# Autodesk Inventor assembly: Shooter Assembly v2
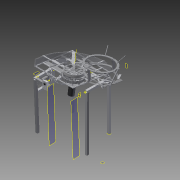
[picture p0: Inventor's stored thumbnail of the model, 180x180]
Saved by Autodesk Inventor 2013 (Build 170138000, 138)
## iProperties
Created: 2013-01-15
Part Number: Shooter Assembly v2
Document SubType Name: Assembly
Designer: actoennies
Mass: 8056.1 g
Surface Area: 23883.9 cm^2
Volume: 3889.96 cm^3
Density: 2.071 g/cm^3
Author: actoennies
## Documents named in this file (34)
- \\NNHSSRV2.hs.sd203.org\ACToennies$\Robotics\Shooter\Shooter Assembly v2.iam
- \\NNHSSRV2.hs.sd203.org\ACToennies$\Robotics\Shooter\Bearing Mount v1.ipt
- \\NNHSSRV2.hs.sd203.org\ACToennies$\Robotics\Shooter\Outer Rail v1.ipt
- \\NNHSSRV2.hs.sd203.org\ACToennies$\Robotics\Shooter\Runner Rails v2.ipt
- \\NNHSSRV2.hs.sd203.org\ACToennies$\Robotics\Shooter\Bearing.ipt
- \\NNHSSRV2.hs.sd203.org\ACToennies$\Robotics\Shooter\Flywheel Assembly.iam
- \\NNHSSRV2.hs.sd203.org\ACToennies$\Robotics\Shooter\Shooter Mounter.ipt
- \\NNHSSRV2.hs.sd203.org\ACToennies$\Robotics\Shooter\Bearing Mount 2 v1.ipt
- \\NNHSSRV2.hs.sd203.org\ACToennies$\Robotics\Shooter\Shorter Shaft.ipt
- \\NNHSSRV2.hs.sd203.org\ACToennies$\Robotics\Shooter\Spacer Rube.ipt
- \\NNHSSRV2.hs.sd203.org\ACToennies$\Robotics\Shooter\Edge Mount.ipt
- \\NNHSSRV2.hs.sd203.org\ACToennies$\Robotics\Shooter\Tower Corner Mount.ipt
- \\NNHSSRV2.hs.sd203.org\ACToennies$\Robotics\Shooter\Square Tube.ipt
- \\NNHSSRV2.hs.sd203.org\ACToennies$\Robotics\Shooter\Flange Bearing Mount Tower.ipt
- \\NNHSSRV2.hs.sd203.org\ACToennies$\Robotics\Shooter\Flange Bearing Mount Tower Mirror.ipt
- \\NNHSSRV2.hs.sd203.org\ACToennies$\Robotics\Shooter\Bearing Mount Top.ipt
- \\NNHSSRV2.hs.sd203.org\ACToennies$\Robotics\Shooter\Square Motor Mount.ipt
- \\NNHSSRV2.hs.sd203.org\ACToennies$\Robotics\Hopper\HopperAssembly42inch_v5.iam
- \\NNHSSRV2.hs.sd203.org\ACToennies$\Robotics\Shooter\Shooter Assembly v2\Design Accelerator\Spur Gears1.iam
- \\NNHSSRV2.hs.sd203.org\ACToennies$\Robotics\Parts\Imported Components\Snow Blower Motor\Snow Blower Motor.iam
- \\NNHSSRV2.hs.sd203.org\ACToennies$\Robotics\Shooter\Snowblower Motor Mount.ipt
- \\NNHSSRV2.hs.sd203.org\ACToennies$\Robotics\Shooter\Edge Mount Interference.ipt
- \\NNHSSRV2.hs.sd203.org\ACToennies$\Robotics\Shooter\8mm shaft.ipt
- \\NNHSSRV2.hs.sd203.org\ACToennies$\Robotics\Shooter\CIM Bearing.ipt
- H:\Robotics\Parts\8 Plaction Wheel.iam
- \\NNHSSRV2.hs.sd203.org\ACToennies$\Robotics\Shooter\Square Tube 2.ipt
- \\NNHSSRV2.hs.sd203.org\ACToennies$\Robotics\Parts\CIM Motor\Motors_FR801-001.iam
- \\NNHSSRV2.hs.sd203.org\ACToennies$\Robotics\Shooter\Cim Mount.ipt
- \\NNHSSRV2.hs.sd203.org\ACToennies$\Robotics\Shooter\Hub v1.ipt
- \\NNHSSRV2.hs.sd203.org\ACToennies$\Robotics\Shooter\Camera Traffic Light Mount.ipt
- \\NNHSSRV2.hs.sd203.org\ACToennies$\Robotics\Shooter\Camera Gusset Plat.ipt
- \\NNHSSRV2.hs.sd203.org\ACToennies$\Inventor\Camera.ipt
- \\NNHSSRV2.hs.sd203.org\ACToennies$\Robotics\Shooter\Square Tube 3.ipt
- \\NNHSSRV2.hs.sd203.org\ACToennies$\Robotics\Shooter\Square Tube 4.ipt
## Components (40 placed, 33 different names)
1. Bearing Mount v1:1 — Insert:12, Insert:13, Insert:14, Insert:15, Insert:26, Insert:27, Mate:62, Mate:63
2. Outer Rail v1:1 — Insert:12, Insert:13, Insert:47, Insert:48, Flush:21, Mate:87
3. Runner Rails v2:1 — Insert:14, Insert:15, Mate:42
4. Flywheel Assembly:1 [sub-assembly] — Mate:61, Flush:30, Mate:68, Flush:31
5. Shooter Mounter:1 — Insert:26, Insert:27, Insert:34, Flush:11, Insert:35, Insert:36, Insert:37, Insert:38, Flush:19, Mate:45, Flush:24, Flush:40
6. Spacer Rube:1 — Insert:34, Flush:11
7. Bearing Mount 2 v1:1 — Insert:37, Insert:38, Insert:40
8. Bearing Mount 2 v1:2 — Insert:35, Insert:36, Insert:39
9. Bearing:3 — Insert:40, Flush:13, Mate:14, Mate:15
10. Bearing:4 — Insert:39, Flush:12, Mate:12, Mate:13, Mate:36, Mate:44
11. Shorter Shaft:1 — Flush:12, Mate:12, Mate:13, Mate:37
12. Shorter Shaft:2 — Flush:13, Mate:14, Mate:15, Mate:38
13. Tower Corner Mount:1 — Mate:16, Flush:14, Mate:48, Flush:33
14. Edge Mount:2 — Flush:34, Mate:104, Flush:48, Mate:105, Mate:106, Flush:50
15. Square Tube:2 — Mate:16, Flush:14, Insert:41, Insert:42, Flush:19, Flush:23, Flush:26, Mate:50, Mate:52, Flush:27, Mate:81, Flush:32, Mate:93, Flush:41, Flush:42
16. Flange Bearing Mount Tower:1 — Insert:41, Insert:42, Insert:43
17. Bearing:5 — Insert:43, Mate:36, Mate:37
18. Flange Bearing Mount Tower Mirror:1 — Insert:46, Flush:29
19. Bearing:6 — Insert:46, Mate:38
20. Bearing Mount Top:1 — Insert:47, Insert:48, Mate:65, Mate:66, Mate:68
21. Square Motor Mount:1 — Flush:23, Mate:47, Mate:48, Mate:51, Flush:27, Mate:77
22. HopperAssembly42inch_v5:1 [sub-assembly] — Mate:42, Flush:21, Mate:87
23. Spur Gears:1 [sub-assembly] — Mate:44, Mate:45, Flush:24, Flush:25, Mate:46, Angle:2
24. Snow Blower Motor:1 [sub-assembly] — Flush:25, Mate:46, Angle:2, Insert:50, Insert:51
25. Snowblower Motor Mount:1 — Insert:50, Insert:51, Mate:47, Mate:51, Mate:52
26. Edge Mount Interference:1 — Flush:26, Mate:50, Mate:77, Mate:95, Flush:44, Flush:45, Flush:46
27. 8mm shaft:1 — Mate:61, Flush:30, Mate:67, Flush:31, Mate:82, Mate:83, Mate:84, Mate:86
28. CIM Bearing:1 — Mate:65, Mate:66, Mate:67
29. CIM Bearing:2 — Mate:62, Mate:63, Insert:56
30. 8 Plaction Wheel:1 [sub-assembly] — Mate:88, Mate:89, Mate:90, Mate:91, Mate:92
31. Square Tube 2:1 — Mate:81, Flush:32, Flush:33, Flush:34, Mate:106, Mate:107
32. Motors_FR801-001:1 [sub-assembly] — Mate:82, Mate:83, Mate:84, Insert:58
33. Cim Mount:1 — Insert:58, Flush:40
34. Hub v1:1 — Mate:88, Mate:89, Mate:90, Flush:38
35. Hub v1:2 — Mate:91, Flush:38, Mate:92, Insert:56
36. Camera Traffic Light Mount:1 — Mate:93, Flush:41, Flush:42, Mate:94, Flush:43, Mate:101, Mate:102, Mate:103
37. Camera Gusset Plat:1 — Mate:94, Mate:95, Flush:43
38. Camera:1 — Mate:101, Mate:102, Mate:103
39. Square Tube 3:1 — Mate:104, Flush:48, Mate:105, Mate:107, Mate:109, Mate:110, Mate:112, Mate:113, Mate:117, Mate:121
40. Square Tube 4:1 — Mate:114, Mate:115, Mate:116, Mate:117, Mate:119, Mate:121
## Relationships (108: Mate 57, Flush 27, Insert 23, Angle 1)
- Insert:12: Bearing Mount v1:1 ↔ Outer Rail v1:1
- Insert:13: Bearing Mount v1:1 ↔ Outer Rail v1:1
- Insert:14: Bearing Mount v1:1 ↔ Runner Rails v2:1
- Insert:15: Bearing Mount v1:1 ↔ Runner Rails v2:1
- Insert:26: Bearing Mount v1:1 ↔ Shooter Mounter:1
- Insert:27: Bearing Mount v1:1 ↔ Shooter Mounter:1
- Insert:34: Shooter Mounter:1 ↔ Spacer Rube:1
- Flush:11: Shooter Mounter:1 ↔ Spacer Rube:1
- Insert:35: Shooter Mounter:1 ↔ Bearing Mount 2 v1:2
- Insert:36: Shooter Mounter:1 ↔ Bearing Mount 2 v1:2
- Insert:37: Shooter Mounter:1 ↔ Bearing Mount 2 v1:1
- Insert:38: Shooter Mounter:1 ↔ Bearing Mount 2 v1:1
- Insert:39: Bearing Mount 2 v1:2 ↔ Bearing:4
- Insert:40: Bearing Mount 2 v1:1 ↔ Bearing:3
- Flush:12 (-25.4 mm): Bearing:4 ↔ Shorter Shaft:1
- Mate:12: Bearing:4 ↔ Shorter Shaft:1
- Mate:13: Bearing:4 ↔ Shorter Shaft:1
- Flush:13 (-25.4 mm): Bearing:3 ↔ Shorter Shaft:2
- Mate:14: Bearing:3 ↔ Shorter Shaft:2
- Mate:15: Bearing:3 ↔ Shorter Shaft:2
- Mate:16: Tower Corner Mount:1 ↔ Square Tube:2
- Flush:14: Tower Corner Mount:1 ↔ Square Tube:2
- Insert:41: Square Tube:2 ↔ Flange Bearing Mount Tower:1
- Insert:42: Square Tube:2 ↔ Flange Bearing Mount Tower:1
- Insert:43: Flange Bearing Mount Tower:1 ↔ Bearing:5
- Flush:19: Shooter Mounter:1 ↔ Square Tube:2
- Mate:36: Bearing:4 ↔ Bearing:5
- Mate:37: Shorter Shaft:1 ↔ Bearing:5
- Insert:46: Flange Bearing Mount Tower Mirror:1 ↔ Bearing:6
- Mate:38: Shorter Shaft:2 ↔ Bearing:6
- Insert:47: Outer Rail v1:1 ↔ Bearing Mount Top:1
- Insert:48: Outer Rail v1:1 ↔ Bearing Mount Top:1
- Mate:42: Runner Rails v2:1 ↔ HopperAssembly42inch_v5:1
- Flush:21: Outer Rail v1:1 ↔ HopperAssembly42inch_v5:1
- Flush:23 (152.4 mm): Square Tube:2 ↔ Square Motor Mount:1
- Mate:44: Bearing:4 ↔ Spur Gears:1
- Mate:45 (25.4 mm): Shooter Mounter:1 ↔ Spur Gears:1
- Flush:24: Shooter Mounter:1 ↔ Spur Gears:1
- Flush:25 (-3.175 mm): Spur Gears:1 ↔ Snow Blower Motor:1
- Mate:46: Spur Gears:1 ↔ Snow Blower Motor:1
- Angle:2 (0 deg): Spur Gears:1 ↔ Snow Blower Motor:1
- Insert:50: Snow Blower Motor:1 ↔ Snowblower Motor Mount:1
- Insert:51: Snow Blower Motor:1 ↔ Snowblower Motor Mount:1
- Mate:47: Square Motor Mount:1 ↔ Snowblower Motor Mount:1
- Mate:48: Tower Corner Mount:1 ↔ Square Motor Mount:1
- Flush:26: Square Tube:2 ↔ Edge Mount Interference:1
- Mate:50: Square Tube:2 ↔ Edge Mount Interference:1
- Mate:51: Square Motor Mount:1 ↔ Snowblower Motor Mount:1
- Mate:52: Square Tube:2 ↔ Snowblower Motor Mount:1
- Flush:27: Square Tube:2 ↔ Square Motor Mount:1
- Flush:29 (203.2 mm): Flange Bearing Mount Tower Mirror:1
- Mate:61: Flywheel Assembly:1 ↔ 8mm shaft:1
- Flush:30 (12.7 mm): Flywheel Assembly:1 ↔ 8mm shaft:1
- Mate:62: Bearing Mount v1:1 ↔ CIM Bearing:2
- Mate:63: Bearing Mount v1:1 ↔ CIM Bearing:2
- Mate:65: Bearing Mount Top:1 ↔ CIM Bearing:1
- Mate:66: Bearing Mount Top:1 ↔ CIM Bearing:1
- Mate:67: 8mm shaft:1 ↔ CIM Bearing:1
- Mate:68 (6.35 mm): Flywheel Assembly:1 ↔ Bearing Mount Top:1
- Flush:31: Flywheel Assembly:1 ↔ 8mm shaft:1
- Mate:77: Square Motor Mount:1 ↔ Edge Mount Interference:1
- Mate:81: Square Tube:2 ↔ Square Tube 2:1
- Flush:32: Square Tube:2 ↔ Square Tube 2:1
- Flush:33: Tower Corner Mount:1 ↔ Square Tube 2:1
- Flush:34: Edge Mount:2 ↔ Square Tube 2:1
- Mate:82: 8mm shaft:1 ↔ Motors_FR801-001:1
- Mate:83: 8mm shaft:1 ↔ Motors_FR801-001:1
- Mate:84: 8mm shaft:1 ↔ Motors_FR801-001:1
- Mate:86: 8mm shaft:1
- Mate:87 (25.4 mm): Outer Rail v1:1 ↔ HopperAssembly42inch_v5:1
- Mate:88: 8 Plaction Wheel:1 ↔ Hub v1:1
- Mate:89: 8 Plaction Wheel:1 ↔ Hub v1:1
- Mate:90: 8 Plaction Wheel:1 ↔ Hub v1:1
- Mate:91: 8 Plaction Wheel:1 ↔ Hub v1:2
- Flush:38: Hub v1:1 ↔ Hub v1:2
- Mate:92: 8 Plaction Wheel:1 ↔ Hub v1:2
- Insert:56 (3.175 mm): CIM Bearing:2 ↔ Hub v1:2
- Insert:58: Motors_FR801-001:1 ↔ Cim Mount:1
- Flush:40: Shooter Mounter:1 ↔ Cim Mount:1
- Mate:93: Square Tube:2 ↔ Camera Traffic Light Mount:1
- Flush:41: Square Tube:2 ↔ Camera Traffic Light Mount:1
- Flush:42: Square Tube:2 ↔ Camera Traffic Light Mount:1
- Mate:94: Camera Traffic Light Mount:1 ↔ Camera Gusset Plat:1
- Mate:95: Edge Mount Interference:1 ↔ Camera Gusset Plat:1
- Flush:43 (11.1125 mm): Camera Traffic Light Mount:1 ↔ Camera Gusset Plat:1
- Flush:44 (-203.2 mm): Edge Mount Interference:1
- Flush:45 (-508 mm): Edge Mount Interference:1
- Flush:46 (-660.4 mm): Edge Mount Interference:1
- Mate:101: Camera Traffic Light Mount:1 ↔ Camera:1
- Mate:102: Camera Traffic Light Mount:1 ↔ Camera:1
- Mate:103: Camera Traffic Light Mount:1 ↔ Camera:1
- Mate:104: Edge Mount:2 ↔ Square Tube 3:1
- Flush:48: Edge Mount:2 ↔ Square Tube 3:1
- Mate:105: Edge Mount:2 ↔ Square Tube 3:1
- Mate:106: Edge Mount:2 ↔ Square Tube 2:1
- Mate:107: Square Tube 2:1 ↔ Square Tube 3:1
- Mate:109: Square Tube 3:1
- Mate:110: Square Tube 3:1
- Mate:112: Square Tube 3:1
- Mate:113: Square Tube 3:1
- Flush:50: Edge Mount:2
- Mate:114: Square Tube 4:1
- Mate:115: Square Tube 4:1
- Mate:116: Square Tube 4:1
- Mate:117: Square Tube 3:1 ↔ Square Tube 4:1
- Mate:119: Square Tube 4:1
- Mate:120
- Mate:121: Square Tube 3:1 ↔ Square Tube 4:1
